# Autodesk Inventor assembly: asstseal
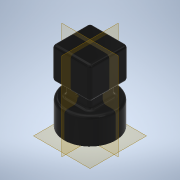
[picture p0: Inventor's stored thumbnail of the model, 180x180]
Saved by Autodesk Inventor 2020.3 (Build 243373000, 373)
## iProperties
Created: 2020-10-22
Part Number: asstseal
Material: 一般
Document SubType Name: Assembly
Designer: Masato
Author: Masato
## Documents named in this file (3)
- C:\Users\masato\Documents\GitHub\設計製作論3\colorseal_model\asstseal.iam
- C:\Users\masato\Documents\GitHub\設計製作論3\colorseal_model\asst.ipt
- C:\Users\masato\Documents\GitHub\設計製作論3\colorseal_model\seal.ipt
## Components (2 placed, 2 different names)
1. asst:1 — 挿入:1, 角度:1, メイト:2, メイト:3
2. seal:1 — 挿入:1, 角度:1, メイト:4
## Relationships (5: Mate 3, Insert 1, Angle 1)
- 挿入:1 [Insert]: asst:1 ↔ seal:1
- 角度:1 [Angle] (0 deg): asst:1 ↔ seal:1
- メイト:2 [Mate] (-15 mm): asst:1
- メイト:3 [Mate] (-15 mm): asst:1
- メイト:4 [Mate]: seal:1
